# Autodesk Inventor assembly: Сервопривод с кареткой
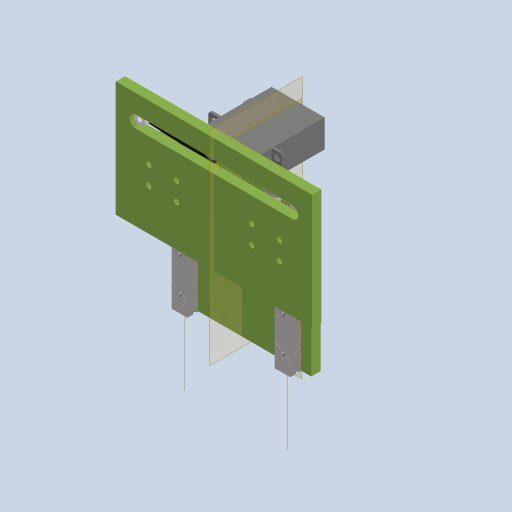
[picture p0: Inventor's stored thumbnail of the model, 512x512]
Saved by Autodesk Inventor 2024.2 (Build 282272000, 272)
## iProperties
Created: 2025-11-27
Part Number: Сервопривод с кареткой
Document SubType Name: Assembly
Designer: katya_notebook
Author: katya_notebook
## Documents named in this file (10)
- C:\Users\91125\OneDrive\Рабочий стол\alletz\3д модель\Сервопривод с кареткой.iam
- C:\Users\91125\OneDrive\Рабочий стол\alletz\3д модель\JX Servo PDI-HV2006MG\JX Servo PDI-HV2006MG.ipt
- C:\Users\91125\OneDrive\Рабочий стол\alletz\3д модель\MGN7C каретка\MGN7C каретка.ipt
- C:\Users\91125\OneDrive\Рабочий стол\alletz\3д модель\MHN7C рельса\MHN7C рельса.ipt
- C:\Users\91125\OneDrive\Рабочий стол\alletz\3д модель\крепление рельс.ipt
- C:\Users\91125\OneDrive\Рабочий стол\alletz\3д модель\крепление каретки.ipt
- C:\Users\91125\OneDrive\Рабочий стол\alletz\3д модель\подшипник мини.ipt
- C:\Users\91125\OneDrive\Рабочий стол\alletz\3д модель\деталь которая двигает.ipt
- C:\Users\91125\OneDrive\Рабочий стол\alletz\3д модель\деталь на которой рельсы.ipt
- C:\Users\91125\OneDrive\Рабочий стол\alletz\3д модель\25T Servo Horn Steering Arm M3 версия 3.ipt
## Components (11 placed, 9 different names)
1. JX Servo PDI-HV2006MG:1 — Совмещение:5, Совмещение:9, Совмещение:10, С поворотом:1, Совмещение:11
2. MGN7C каретка:1 — Жесткий:2, Совмещение:8
3. MHN7C рельса:1 — Совмещение:2, Заподлицо:1, Совмещение:3, Совмещение:4, Жесткий:2, Совмещение:6, Совмещение:7, Заподлицо:3
4. крепление рельс:1
5. крепление каретки:1
6. подшипник мини:1 — Совмещение:12
7. MHN7C рельса:2 — Заподлицо:1, Совмещение:3, Совмещение:6, Совмещение:7, Жесткий:3
8. MGN7C каретка:2 — Жесткий:3, Совмещение:8, Заподлицо:4, Совмещение:11
9. деталь которая двигает:1 — Заподлицо:3
10. деталь на которой рельсы:1 — Заподлицо:4, Совмещение:9
11. 25T Servo Horn Steering Arm M3 версия 3:1 — Совмещение:10, С поворотом:1, Совмещение:12
## Relationships (17: Mate 11, Flush 3, WeldJoint 2, RevoluteJoint 1)
- Совмещение:2 [Mate]: MHN7C рельса:1
- Заподлицо:1 [Flush]: MHN7C рельса:1 ↔ MHN7C рельса:2
- Совмещение:3 [Mate] (38 mm): MHN7C рельса:1 ↔ MHN7C рельса:2
- Совмещение:4 [Mate] (22.3 mm): MHN7C рельса:1
- Совмещение:5 [Mate]: JX Servo PDI-HV2006MG:1
- Жесткий:2 [WeldJoint]: MGN7C каретка:1 ↔ MHN7C рельса:1
- Совмещение:6 [Mate]: MHN7C рельса:1 ↔ MHN7C рельса:2
- Совмещение:7 [Mate]: MHN7C рельса:1 ↔ MHN7C рельса:2
- Жесткий:3 [WeldJoint]: MHN7C рельса:2 ↔ MGN7C каретка:2
- Совмещение:8 [Mate]: MGN7C каретка:1 ↔ MGN7C каретка:2
- Заподлицо:3 [Flush]: MHN7C рельса:1 ↔ деталь которая двигает:1
- Заподлицо:4 [Flush]: MGN7C каретка:2 ↔ деталь на которой рельсы:1
- Совмещение:9 [Mate] (4.5 mm): JX Servo PDI-HV2006MG:1 ↔ деталь на которой рельсы:1
- Совмещение:10 [Mate]: JX Servo PDI-HV2006MG:1 ↔ 25T Servo Horn Steering Arm M3 версия 3:1
- С поворотом:1 [RevoluteJoint]: JX Servo PDI-HV2006MG:1 ↔ 25T Servo Horn Steering Arm M3 версия 3:1
- Совмещение:11 [Mate]: JX Servo PDI-HV2006MG:1 ↔ MGN7C каретка:2
- Совмещение:12 [Mate]: подшипник мини:1 ↔ 25T Servo Horn Steering Arm M3 версия 3:1
